# Autodesk Inventor assembly: J005097
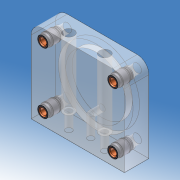
[picture p0: Inventor's stored thumbnail of the model, 180x180]
Saved by Autodesk Inventor 2015 SP1 (Build 190203100, 203)
## iProperties
Created: 2015-03-14
Vendor: HHMI: JRC - ID&F
Document SubType Name: Assembly
Designer: JORDANJ
Project: P-171601
Part Number: J005097
Description: COMPONENT OF AN AUTOMATED LIQUID HANDLING MACHINE SPECIFICALLY DESIGNED FOR THE IN SITU RNA HYBRIDIZATION OF DROSOPHILA EMBRYOS
RuleStatus: InUse
AfterDocSave0: file://Part Number Cleaner
DESIGN DEPARTMENT: HHMI: JRC - ID&F
LAB/DEPT: STERN (LAB)
REQUESTING SCIENTIST: STERN, DAVID
SPECIAL FINISH: POLISH CLEAR
SURFACE ROUGHNESS: 32 Ra
ALTERED ITEM PART NUMBER: N/A
ALTERED ITEM VENDOR: N/A
ALTERED ITEM DESCRIPTION: N/A
Revision Number: -
## Documents named in this file (3)
- C:\_WORKSPACE\DATA\PROJECTS\HYBRIDIZER\MCAD\MICROPLATE\24W SYSTEM SYRINGE BASE.iam
- C:\_WORKSPACE\DATA\PROJECTS\HYBRIDIZER\MCAD\MICROPLATE\24W SYSTEM SYRINGE BASE.ipt
- C:\_WORKSPACE\DATA\Imported Components\20150327-142204-70136782\PEM ISC-832.ipt
## Components (5 placed, 2 different names)
1. 24W SYSTEM SYRINGE BASE:1 — Flush:1, Flush:2, Flush:3, Insert:1, Insert:2, Insert:3, Insert:4
2. PEM ISC-832:1 — Insert:1
3. PEM ISC-832:2 — Insert:2
4. PEM ISC-832:3 — Insert:3
5. PEM ISC-832:4 — Insert:4
## Relationships (7: Insert 4, Flush 3)
- Flush:1: 24W SYSTEM SYRINGE BASE:1
- Flush:2: 24W SYSTEM SYRINGE BASE:1
- Flush:3: 24W SYSTEM SYRINGE BASE:1
- Insert:1: 24W SYSTEM SYRINGE BASE:1 ↔ PEM ISC-832:1
- Insert:2: 24W SYSTEM SYRINGE BASE:1 ↔ PEM ISC-832:2
- Insert:3: 24W SYSTEM SYRINGE BASE:1 ↔ PEM ISC-832:3
- Insert:4: 24W SYSTEM SYRINGE BASE:1 ↔ PEM ISC-832:4
